# Autodesk Inventor assembly: Line Sensor 2 Attachment Assembly
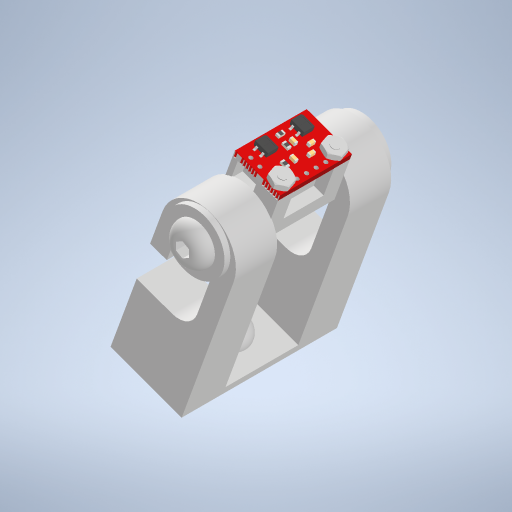
[picture p0: Inventor's stored thumbnail of the model, 512x512]
Saved by Autodesk Inventor 2024 (Build 280153000, 153)
## iProperties
Created: 2023-10-22
Part Number: Line Sensor 2 Attachment Assembly
Document SubType Name: Assembly
Designer: olson
Author: olson
## Documents named in this file (8)
- C:\Users\olson\OneDrive\Documents\Senior Year\FALL 2023\ECE 4961 - Capstone 1\Detial Design\Attachments\CAD\Line Sensor 2 Attachment Assembly.iam
- C:\Users\olson\OneDrive\Documents\Senior Year\FALL 2023\ECE 4961 - Capstone 1\Detial Design\Attachments\CAD\2 Backet Adjustment.ipt
- C:\Users\olson\OneDrive\Documents\Senior Year\FALL 2023\ECE 4961 - Capstone 1\Detial Design\Attachments\CAD\Line Sensor 2 Bracket.ipt
- C:\Users\olson\OneDrive\Documents\Senior Year\FALL 2023\ECE 4961 - Capstone 1\Detial Design\Attachments\CAD\qtr-2rc-reflectance-sensor-array.ipt
- C:\Users\olson\OneDrive\Documents\Senior Year\FALL 2023\ECE 4961 - Capstone 1\Detial Design\Attachments\CAD\1-4 washer.ipt
- C:\Users\olson\OneDrive\Documents\Senior Year\FALL 2023\ECE 4961 - Capstone 1\Detial Design\Attachments\CAD\1-4-20 screw.ipt
- C:\Users\olson\OneDrive\Documents\Senior Year\FALL 2023\ECE 4961 - Capstone 1\Detial Design\Attachments\CAD\2-56 nut.ipt
- C:\Users\olson\OneDrive\Documents\Senior Year\FALL 2023\ECE 4961 - Capstone 1\Detial Design\Attachments\CAD\2-56 screw.ipt
## Components (12 placed, 7 different names)
1. 2 Backet Adjustment:1 — Rotational:5, Rotational:9, Rotational:10, Angle:1
2. 1-4 washer:1 — Rotational:5, Rotational:6
3. 1-4 washer:2 — Rotational:10, Rotational:11, Cylindrical:1
4. 1-4-20 screw:1 — Rotational:6
5. 1-4-20 screw:2 — Rotational:9
6. 1-4-20 screw:3 — Rotational:11
7. 2-56 nut:1 — Rotational:15
8. 2-56 nut:2 — Rotational:14
9. 2-56 screw:1 — Rotational:13
10. 2-56 screw:2 — Rotational:12
11. Line Sensor 2 Bracket:1 — Cylindrical:1, Angle:1, Flush:1, Flush:2, Mate:1, Rotational:12, Rotational:13
12. qtr-2rc-reflectance-sensor-array:1 — Flush:1, Flush:2, Mate:1, Rotational:14, Rotational:15
## Relationships (14: RevoluteJoint 9, Flush 2, CylindricalJoint 1, Angle 1, Mate 1)
- Rotational:5 [RevoluteJoint]: 2 Backet Adjustment:1 ↔ 1-4 washer:1
- Rotational:6 [RevoluteJoint]: 1-4 washer:1 ↔ 1-4-20 screw:1
- Rotational:9 [RevoluteJoint]: 2 Backet Adjustment:1 ↔ 1-4-20 screw:2
- Rotational:10 [RevoluteJoint]: 2 Backet Adjustment:1 ↔ 1-4 washer:2
- Rotational:11 [RevoluteJoint]: 1-4 washer:2 ↔ 1-4-20 screw:3
- Cylindrical:1: 1-4 washer:2 ↔ Line Sensor 2 Bracket:1
- Angle:1 (90 deg): 2 Backet Adjustment:1 ↔ Line Sensor 2 Bracket:1
- Flush:1: Line Sensor 2 Bracket:1 ↔ qtr-2rc-reflectance-sensor-array:1
- Flush:2: Line Sensor 2 Bracket:1 ↔ qtr-2rc-reflectance-sensor-array:1
- Mate:1: Line Sensor 2 Bracket:1 ↔ qtr-2rc-reflectance-sensor-array:1
- Rotational:12 [RevoluteJoint]: 2-56 screw:2 ↔ Line Sensor 2 Bracket:1
- Rotational:13 [RevoluteJoint]: 2-56 screw:1 ↔ Line Sensor 2 Bracket:1
- Rotational:14 [RevoluteJoint]: 2-56 nut:2 ↔ qtr-2rc-reflectance-sensor-array:1
- Rotational:15 [RevoluteJoint]: 2-56 nut:1 ↔ qtr-2rc-reflectance-sensor-array:1
